# Autodesk Inventor assembly: Track Design 9-24-19
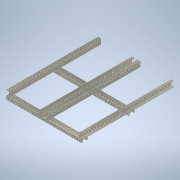
[picture p0: Inventor's stored thumbnail of the model, 180x180]
Saved by Autodesk Inventor 2020 (Build 240168000, 168)
## iProperties
Created: 2019-07-25
Part Number: Track Design 9-24-19
Document SubType Name: Assembly
Designer: Corey
Author: Corey
## Documents named in this file (4)
- C:\Users\Corey\Documents\Tower-Takeover-CAD\Parts\Dual Track.iam
- C:\Users\Corey\Documents\Tower-Takeover-CAD\Parts\Structure\C-Channels\Aluminum\2-Wide\Aluminum C-Channel 1x2x1x35.ipt
- C:\Users\Corey\Documents\Tower-Takeover-CAD\Parts\Structure\C-Channels\Aluminum\2-Wide\Aluminum C-Channel 1x2x1x29.ipt
- C:\Users\Corey\Documents\Tower-Takeover-CAD\Parts\Structure\C-Channels\Aluminum\2-Wide\Aluminum C-Channel 1x2x1x14.ipt
## Components (8 placed, 3 different names)
1. Aluminum C-Channel 1x2x1x35:2 — Flush:24, Mate:10, Flush:25, Flush:26
2. Aluminum C-Channel 1x2x1x35:3
3. Aluminum C-Channel 1x2x1x35:4 — Mate:9
4. Aluminum C-Channel 1x2x1x35:5 — Mate:8, Flush:22, Flush:23, Mate:11, Flush:27, Flush:28
5. Aluminum C-Channel 1x2x1x29:1 — Mate:8, Flush:22, Flush:23
6. Aluminum C-Channel 1x2x1x29:3 — Mate:9, Flush:24
7. Aluminum C-Channel 1x2x1x14:1 — Mate:10, Flush:25, Flush:26
8. Aluminum C-Channel 1x2x1x14:2 — Mate:11, Flush:27, Flush:28
## Relationships (11: Flush 7, Mate 4)
- Mate:8: Aluminum C-Channel 1x2x1x35:5 ↔ Aluminum C-Channel 1x2x1x29:1
- Flush:22: Aluminum C-Channel 1x2x1x35:5 ↔ Aluminum C-Channel 1x2x1x29:1
- Flush:23: Aluminum C-Channel 1x2x1x35:5 ↔ Aluminum C-Channel 1x2x1x29:1
- Mate:9: Aluminum C-Channel 1x2x1x35:4 ↔ Aluminum C-Channel 1x2x1x29:3
- Flush:24: Aluminum C-Channel 1x2x1x35:2 ↔ Aluminum C-Channel 1x2x1x29:3
- Mate:10: Aluminum C-Channel 1x2x1x35:2 ↔ Aluminum C-Channel 1x2x1x14:1
- Mate:11: Aluminum C-Channel 1x2x1x35:5 ↔ Aluminum C-Channel 1x2x1x14:2
- Flush:25: Aluminum C-Channel 1x2x1x35:2 ↔ Aluminum C-Channel 1x2x1x14:1
- Flush:26: Aluminum C-Channel 1x2x1x35:2 ↔ Aluminum C-Channel 1x2x1x14:1
- Flush:27: Aluminum C-Channel 1x2x1x35:5 ↔ Aluminum C-Channel 1x2x1x14:2
- Flush:28: Aluminum C-Channel 1x2x1x35:5 ↔ Aluminum C-Channel 1x2x1x14:2
